# Autodesk Inventor assembly: WheelWithBearing
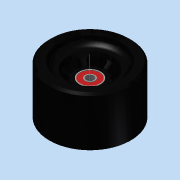
[picture p0: Inventor's stored thumbnail of the model, 180x180]
Saved by Autodesk Inventor 2015 (Build 190159000, 159)
## iProperties
Created: 2015-11-06
Part Number: WheelWithBearing
Document SubType Name: Assembly
Designer: Raphael
Author: Raphael
## Documents named in this file (3)
- \\psf\Home\Documents\electric-skateboard\CAD\WheelWithBearing.iam
- \\psf\Home\Documents\electric-skateboard\CAD\Wheel.ipt
- \\psf\Home\Documents\electric-skateboard\CAD\608Bearing.ipt
## Components (3 placed, 2 different names)
1. Wheel:1 — Mate:1, Mate:2, Mate:3, Mate:4
2. 608Bearing:1 — Mate:1, Mate:3
3. 608Bearing:2 — Mate:2, Mate:4
## Relationships (4: Mate 4)
- Mate:1: Wheel:1 ↔ 608Bearing:1
- Mate:2: Wheel:1 ↔ 608Bearing:2
- Mate:3: Wheel:1 ↔ 608Bearing:1
- Mate:4: Wheel:1 ↔ 608Bearing:2
